# Autodesk Inventor assembly: Сборка1
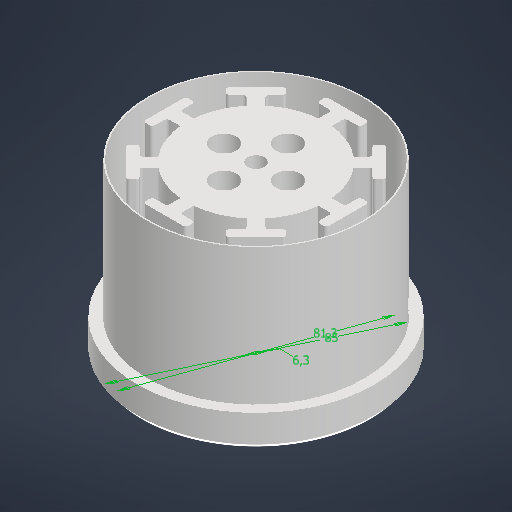
[picture p0: Inventor's stored thumbnail of the model, 512x512]
Saved by Autodesk Inventor 2026.2 (Build 302298000, 298)
## iProperties
Created: 2026-01-09
Part Number: Сборка1
Document SubType Name: Assembly
Designer: Phantom
Author: Phantom
## Documents named in this file (4)
- C:\Users\Phantom\Desktop\Phantom16950\Сборка1.iam
- C:\Users\Phantom\Desktop\24926\Работы Arty\Жопка.ipt
- C:\Users\Phantom\Desktop\24926\Работы Arty\Сердцевина Сиськи.ipt
- C:\Users\Phantom\Desktop\24926\Работы Arty\Округ.ipt
## Components (3 placed, 3 different names)
1. Жопка:1 — Совмещение:1, Совмещение:2, Совмещение:3, Совмещение:4
2. Сердцевина Сиськи:1 — Совмещение:3, Совмещение:4
3. Округ:1 — Совмещение:1, Совмещение:2
## Relationships (4: Mate 4)
- Совмещение:1 [Mate]: Жопка:1 ↔ Округ:1
- Совмещение:2 [Mate]: Жопка:1 ↔ Округ:1
- Совмещение:3 [Mate]: Жопка:1 ↔ Сердцевина Сиськи:1
- Совмещение:4 [Mate]: Жопка:1 ↔ Сердцевина Сиськи:1
